# Autodesk Inventor assembly: bedboltassembly
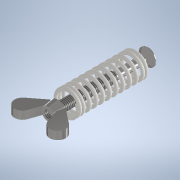
[picture p0: Inventor's stored thumbnail of the model, 180x180]
Saved by Autodesk Inventor 2020.2 (Build 242310000, 310)
## iProperties
Created: 2020-08-25
Part Number: bedboltassembly
Document SubType Name: Assembly
Designer: JK
Author: JK
## Documents named in this file (4)
- C:\Users\JK\Documents\Inventor\Anet Upgrade\bedboltassembly.iam
- C:\Users\JK\Documents\Inventor\Anet Upgrade\bedspring.ipt
- C:\Users\JK\Documents\Inventor\Anet Upgrade\KS B 1014 - M 3.ipt
- C:\Users\JK\Documents\Inventor\Anet Upgrade\AS 1427 - M3 x 30(6) I.ipt
## Components (3 placed, 3 different names)
1. Sprężyna naciskowa1:1 — Mate:1
2. KS B 1014 - Metryczny M 3:1 — Mate:2
3. BS 4183 Wkręt z łbem płaskim wpuszczanym z wgłębieniem krzyżowym do części metalowych - Metryczny M3 x 30:1 — Mate:1, Mate:2
## Relationships (2: Mate 2)
- Mate:1: Sprężyna naciskowa1:1 ↔ BS 4183 Wkręt z łbem płaskim wpuszczanym z wgłębieniem krzyżowym do części metalowych - Metryczny M3 x 30:1
- Mate:2: KS B 1014 - Metryczny M 3:1 ↔ BS 4183 Wkręt z łbem płaskim wpuszczanym z wgłębieniem krzyżowym do części metalowych - Metryczny M3 x 30:1
